# Autodesk Inventor assembly: сборка драйверов_MIR2
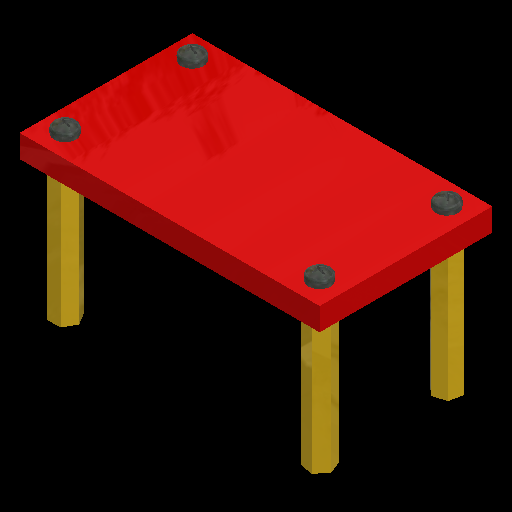
[picture p0: Inventor's stored thumbnail of the model, 512x512]
Saved by Autodesk Inventor 2025 (Build 290162000, 162)
## iProperties
Created: 2025-03-03
Part Number: сборка драйверов_MIR2
Document SubType Name: Assembly
Designer: volko
Mass: 35.1177 g
Surface Area: 97.7601 cm^2
Volume: 15.1248 cm^3
Density: 2.32187 g/cm^3
Author: volko
## Documents named in this file (4)
- C:\Users\volko\Desktop\диплом\Модели\детали\сборка драйверов_MIR2.iam
- C:\Users\volko\Desktop\диплом\Модели\детали\драйвер двигателя_MIR2.ipt
- C:\Users\volko\Desktop\диплом\Модели\детали\втулки крепления электроники_MIR2.ipt
- C:\Users\volko\Desktop\диплом\Модели\детали\стандартные изделия\ru-RU\ISO 7045  H\ISO 7045 - M2,5 x 8_ - 4.8 - H - ISO.ipt
## Components (9 placed, 3 different names)
1. драйвер двигателя_MIR2:1 — Заподлицо:3, Заподлицо:2, Заподлицо:1, Совмещение:5, Совмещение:1, Совмещение:7, Совмещение:2, Совмещение:8, Совмещение:3, Совмещение:6, Совмещение:4, Совмещение:16, Совмещение:12, Совмещение:15, Совмещение:14, Совмещение:13, Совмещение:11
2. втулки крепления электроники_MIR2:1 — Совмещение:5, Совмещение:1, Совмещение:9
3. втулки крепления электроники_MIR2:2 — Совмещение:7, Совмещение:2
4. втулки крепления электроники_MIR2:3 — Совмещение:8, Совмещение:3
5. втулки крепления электроники_MIR2:4 — Совмещение:6, Совмещение:4, Совмещение:10
6. ISO 7045 H M2,5 x 8 - 4.8 - H:1 — Совмещение:16, Совмещение:12
7. ISO 7045 H M2,5 x 8 - 4.8 - H:2 — Совмещение:15, Совмещение:9
8. ISO 7045 H M2,5 x 8 - 4.8 - H:3 — Совмещение:14, Совмещение:10
9. ISO 7045 H M2,5 x 8 - 4.8 - H:4 — Совмещение:13, Совмещение:11
## Relationships (19: Mate 16, Flush 3)
- Заподлицо:3 [Flush]: драйвер двигателя_MIR2:1
- Заподлицо:2 [Flush]: драйвер двигателя_MIR2:1
- Заподлицо:1 [Flush]: драйвер двигателя_MIR2:1
- Совмещение:5 [Mate]: драйвер двигателя_MIR2:1 ↔ втулки крепления электроники_MIR2:1
- Совмещение:1 [Mate]: драйвер двигателя_MIR2:1 ↔ втулки крепления электроники_MIR2:1
- Совмещение:7 [Mate]: драйвер двигателя_MIR2:1 ↔ втулки крепления электроники_MIR2:2
- Совмещение:2 [Mate]: драйвер двигателя_MIR2:1 ↔ втулки крепления электроники_MIR2:2
- Совмещение:8 [Mate]: драйвер двигателя_MIR2:1 ↔ втулки крепления электроники_MIR2:3
- Совмещение:3 [Mate]: драйвер двигателя_MIR2:1 ↔ втулки крепления электроники_MIR2:3
- Совмещение:6 [Mate]: драйвер двигателя_MIR2:1 ↔ втулки крепления электроники_MIR2:4
- Совмещение:4 [Mate]: драйвер двигателя_MIR2:1 ↔ втулки крепления электроники_MIR2:4
- Совмещение:16 [Mate]: драйвер двигателя_MIR2:1 ↔ ISO 7045 H M2,5 x 8 - 4.8 - H:1
- Совмещение:12 [Mate]: драйвер двигателя_MIR2:1 ↔ ISO 7045 H M2,5 x 8 - 4.8 - H:1
- Совмещение:15 [Mate]: драйвер двигателя_MIR2:1 ↔ ISO 7045 H M2,5 x 8 - 4.8 - H:2
- Совмещение:9 [Mate]: втулки крепления электроники_MIR2:1 ↔ ISO 7045 H M2,5 x 8 - 4.8 - H:2
- Совмещение:14 [Mate]: драйвер двигателя_MIR2:1 ↔ ISO 7045 H M2,5 x 8 - 4.8 - H:3
- Совмещение:10 [Mate]: втулки крепления электроники_MIR2:4 ↔ ISO 7045 H M2,5 x 8 - 4.8 - H:3
- Совмещение:13 [Mate]: драйвер двигателя_MIR2:1 ↔ ISO 7045 H M2,5 x 8 - 4.8 - H:4
- Совмещение:11 [Mate]: драйвер двигателя_MIR2:1 ↔ ISO 7045 H M2,5 x 8 - 4.8 - H:4
